# Autodesk Inventor assembly: 00_XY_stage-Chinese_60x60-R1_R1
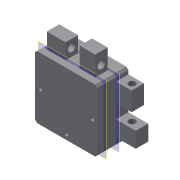
[picture p0: Inventor's stored thumbnail of the model, 180x180]
Saved by Autodesk Inventor 2019 (Build 230136000, 136)
## iProperties
Created: 2019-05-02
Part Number: 00_XY_stage-Chinese_60x60-R1_R1
Document SubType Name: Assembly
Designer: diederichbenedict
Author: diederichbenedict
## Documents named in this file (5)
- C:\Users\diederichbenedict\Dropbox\Dokumente\Promotion\PROJECTS\STORMoChip\INVENTOR\Nanoscopy-on-a-cheap\00_XY_stage-Chinese_60x60-R1_R1.iam
- C:\Users\diederichbenedict\Dropbox\Dokumente\Promotion\PROJECTS\STORMoChip\INVENTOR\Nanoscopy-on-a-cheap\00_XY_stage-Chinese_60x60-R1-Top_R1.ipt
- C:\Users\diederichbenedict\Dropbox\Dokumente\Promotion\PROJECTS\STORMoChip\INVENTOR\Nanoscopy-on-a-cheap\00_XY_stage-Chinese_60x60-R1-Middle_R1.ipt
- C:\Users\diederichbenedict\Dropbox\Dokumente\Promotion\PROJECTS\STORMoChip\INVENTOR\Nanoscopy-on-a-cheap\00_XY_stage-Chinese_60x60-R1-Bottom_R1.ipt
- C:\Users\diederichbenedict\Dropbox\Dokumente\Promotion\PROJECTS\STORMoChip\INVENTOR\Nanoscopy-on-a-cheap\00_XY_stage-CHUO_SEIKI_LD-647-R1-Micrometer_R1.ipt
## Components (5 placed, 4 different names)
1. 00_XY_stage-Chinese_60x60-R1-Top_R1:1 — Flush:2, Flush:1
2. 00_XY_stage-Chinese_60x60-R1-Middle_R1:1 — Flush:2, Flush:1, Flush:4, Flush:3
3. 00_XY_stage-Chinese_60x60-R1-Bottom_R1:1 — Flush:4, Flush:3
4. 00_XY_stage-CHUO_SEIKI_LD-647-R1-Micrometer_R1:1
5. 00_XY_stage-CHUO_SEIKI_LD-647-R1-Micrometer_R1:2
## Relationships (4: Mate 4)
- Flush:2 [Mate]: 00_XY_stage-Chinese_60x60-R1-Top_R1:1 ↔ 00_XY_stage-Chinese_60x60-R1-Middle_R1:1
- Flush:1 [Mate]: 00_XY_stage-Chinese_60x60-R1-Top_R1:1 ↔ 00_XY_stage-Chinese_60x60-R1-Middle_R1:1
- Flush:4 [Mate]: 00_XY_stage-Chinese_60x60-R1-Middle_R1:1 ↔ 00_XY_stage-Chinese_60x60-R1-Bottom_R1:1
- Flush:3 [Mate]: 00_XY_stage-Chinese_60x60-R1-Middle_R1:1 ↔ 00_XY_stage-Chinese_60x60-R1-Bottom_R1:1
